# Autodesk Inventor assembly: Stabilizer_Cherry_MX_2u
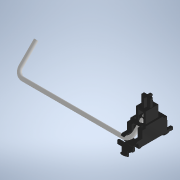
[picture p0: Inventor's stored thumbnail of the model, 180x180]
Saved by Autodesk Inventor 2022 (Build 260153000, 153)
## iProperties
Created: 2021-09-25
Part Number: Stabilizer_Cherry_MX_2u
Document SubType Name: Assembly
Designer: shiok
Author: shiok
## Documents named in this file (3)
- C:\Users\Yazawa\Documents\GitHub\Keyboard_H\pcb\3D_model\step\Stabilizer_Cherry_MX_2u.iam
- C:\Users\Yazawa\Documents\GitHub\Keyboard_H\pcb\3D_model\step\COMPOUND_1.ipt
- C:\Users\Yazawa\Documents\GitHub\Keyboard_H\chassis\2022\stabbar_u5.ipt
## Components (2 placed, 2 different names)
1. 84 — メイト:1, 正接:1, 正接:2, 正接:3
2. stabbar_u5:1 — メイト:1, 正接:1, 正接:2, 正接:3
## Relationships (4: Tangent 3, Mate 1)
- メイト:1 [Mate]: 84 ↔ stabbar_u5:1
- 正接:1 [Tangent]: 84 ↔ stabbar_u5:1
- 正接:2 [Tangent]: 84 ↔ stabbar_u5:1
- 正接:3 [Tangent]: 84 ↔ stabbar_u5:1
